# Autodesk Inventor assembly: Assembly1
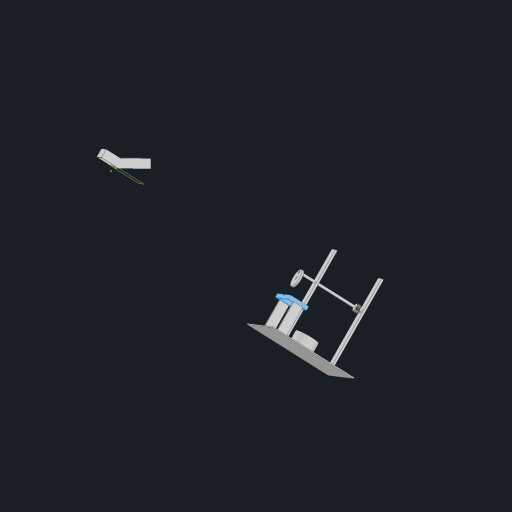
[picture p0: Inventor's stored thumbnail of the model, 512x512]
Saved by Autodesk Inventor 2024 (Build 280153000, 153)
## iProperties
Created: 2023-11-07
Part Number: Assembly1
Document SubType Name: Assembly
Designer: 91840
Author: 91840
## Documents named in this file (10)
- C:\Users\91840\Documents\Inventor\project\Assembly1.iam
- C:\Users\91840\Documents\Inventor\project\base plate.ipt
- C:\Users\91840\Documents\Inventor\project\container.ipt
- C:\Users\91840\Documents\Inventor\project\pillar.ipt
- C:\Users\91840\Documents\Inventor\project\small pillar.ipt
- C:\Users\91840\Documents\Inventor\project\Cutter-bed.ipt
- C:\Users\91840\Documents\Inventor\project\shaft.ipt
- C:\Users\91840\Documents\Inventor\project\disk.ipt
- C:\Users\91840\Documents\Inventor\project\channel.ipt
- C:\Users\91840\Documents\Inventor\practice\project\spur.iam
## Components (11 placed, 9 different names)
1. base plate:1 — Mate:1, Mate:2, Mate:4, Mate:5, Mate:6, Mate:7, Mate:9, Mate:10, Mate:11, Mate:13, Mate:16
2. pillar:1 — Mate:1, Mate:2, Mate:3, Mate:6, Mate:8, Mate:21, Mate:25, Mate:30
3. container:1 — Mate:3, Mate:4, Mate:5
4. pillar:2 — Mate:7, Mate:8, Mate:9, Mate:12, Mate:15, Mate:22
5. small pillar:1 — Mate:10, Mate:11, Mate:12, Mate:17, Mate:18, Mate:19
6. small pillar:2 — Mate:13, Mate:15, Mate:16, Mate:20
7. Cutter-bed:1 — Mate:17, Mate:18, Mate:19, Mate:20, Mate:27
8. shaft:1 — Mate:21, Mate:22, Mate:25, Mate:28, Mate:29, Mate:31
9. disk:1 — Mate:28, Mate:29
10. channel:1 — Mate:27
11. spur:1 [sub-assembly] — Mate:30, Mate:31
## Relationships (27: Mate 27)
- Mate:1 (50 mm): base plate:1 ↔ pillar:1
- Mate:2 (116 mm): base plate:1 ↔ pillar:1
- Mate:3 (160 mm): pillar:1 ↔ container:1
- Mate:4: base plate:1 ↔ container:1
- Mate:5 (-141 mm): base plate:1 ↔ container:1
- Mate:6: base plate:1 ↔ pillar:1
- Mate:7: base plate:1 ↔ pillar:2
- Mate:8 (245 mm): pillar:1 ↔ pillar:2
- Mate:9 (116 mm): base plate:1 ↔ pillar:2
- Mate:10 (-50 mm): base plate:1 ↔ small pillar:1
- Mate:11: base plate:1 ↔ small pillar:1
- Mate:12 (22 mm): pillar:2 ↔ small pillar:1
- Mate:13: base plate:1 ↔ small pillar:2
- Mate:15 (22 mm): pillar:2 ↔ small pillar:2
- Mate:16: base plate:1 ↔ small pillar:2
- Mate:17: small pillar:1 ↔ Cutter-bed:1
- Mate:18: small pillar:1 ↔ Cutter-bed:1
- Mate:19 (75 mm): small pillar:1 ↔ Cutter-bed:1
- Mate:20: small pillar:2 ↔ Cutter-bed:1
- Mate:21: pillar:1 ↔ shaft:1
- Mate:22: pillar:2 ↔ shaft:1
- Mate:25: pillar:1 ↔ shaft:1
- Mate:27: Cutter-bed:1 ↔ channel:1
- Mate:28: shaft:1 ↔ disk:1
- Mate:29 (-10 mm): shaft:1 ↔ disk:1
- Mate:30: pillar:1 ↔ spur:1
- Mate:31: shaft:1 ↔ spur:1
